# Autodesk Inventor assembly: Riemenspanner_Bottompart_Assembly
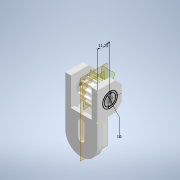
[picture p0: Inventor's stored thumbnail of the model, 180x180]
Saved by Autodesk Inventor 2022 (Build 260153000, 153)
## iProperties
Created: 2022-10-05
Part Number: Riemenspanner_Bottompart_Assembly
Document SubType Name: Assembly
Designer: alexw
Mass: 20.3145 g
Surface Area: 85.039 cm^2
Volume: 10.5826 cm^3
Author: alexw
## Documents named in this file (5)
- C:\Users\AEWALDER\Documents\Inventor\03_CurrentProjects\MasterThesis\PSM_V1_Rillenkugellager\Riemenspanner_Bottompart_Assembly.iam
- C:\Users\AEWALDER\Documents\Inventor\03_CurrentProjects\MasterThesis\PSM_V1_Rillenkugellager\BeltDiscBottomPart.ipt
- C:\Users\AEWALDER\Documents\Inventor\03_CurrentProjects\MasterThesis\PSM_V1_Rillenkugellager\Schaft_6mmx28.5.ipt
- C:\Users\AEWALDER\Documents\Inventor\03_CurrentProjects\MasterThesis\PSM_V1_Rillenkugellager\Vorlage\12TBeltDisc.ipt
- C:\Users\AEWALDER\Documents\Inventor\03_CurrentProjects\MasterThesis\PSM_V1_Rillenkugellager\Maschinenbauteil\SKF_WBB1-8706-2RS1\SKF_WBB1-8706-2RS1.iam
## Components (5 placed, 4 different names)
1. BeltDiscBottomPart:1 — Fluchtend:1, Fluchtend:2, Fluchtend:3, Fluchtend:4, Passend:7, Fluchtend:6, Passend:8, Fluchtend:7, Flush:8
2. SKF_WBB1-8706-2RS1:1 [sub-assembly] — Passend:7, Fluchtend:6
3. SKF_WBB1-8706-2RS1:2 [sub-assembly] — Passend:8, Fluchtend:7, Passend:9
4. Schaft_6mmx28.5:1 — Fluchtend:4, Passend:6, Passend:9
5. 12TBeltDisc:1 — Passend:6, Flush:8
## Relationships (11: Flush 7, Mate 4)
- Fluchtend:1 [Flush]: BeltDiscBottomPart:1
- Fluchtend:2 [Flush]: BeltDiscBottomPart:1
- Fluchtend:3 [Flush]: BeltDiscBottomPart:1
- Fluchtend:4 [Flush]: BeltDiscBottomPart:1 ↔ Schaft_6mmx28.5:1
- Passend:6 [Mate]: Schaft_6mmx28.5:1 ↔ 12TBeltDisc:1
- Passend:7 [Mate]: BeltDiscBottomPart:1 ↔ SKF_WBB1-8706-2RS1:1
- Fluchtend:6 [Flush]: BeltDiscBottomPart:1 ↔ SKF_WBB1-8706-2RS1:1
- Passend:8 [Mate]: BeltDiscBottomPart:1 ↔ SKF_WBB1-8706-2RS1:2
- Fluchtend:7 [Flush]: BeltDiscBottomPart:1 ↔ SKF_WBB1-8706-2RS1:2
- Passend:9 [Mate]: SKF_WBB1-8706-2RS1:2 ↔ Schaft_6mmx28.5:1
- Flush:8: BeltDiscBottomPart:1 ↔ 12TBeltDisc:1
